# Autodesk Inventor assembly: Wheel Assembly
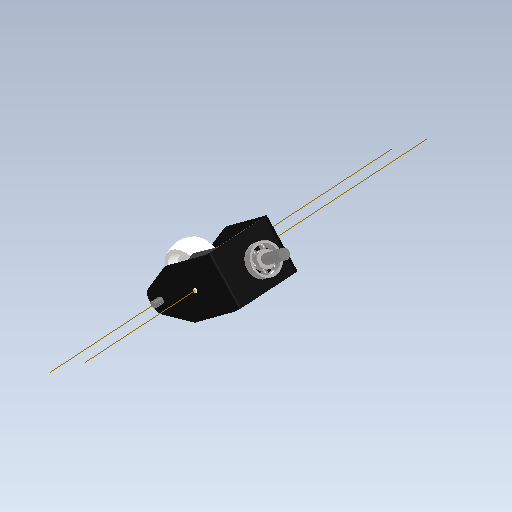
[picture p0: Inventor's stored thumbnail of the model, 512x512]
Saved by Autodesk Inventor 2020 (Build 240168000, 168)
## iProperties
Created: 2022-07-01
Part Number: Wheel Assembly
Document SubType Name: Assembly
Designer: karimi2
Author: karimi2
## Documents named in this file (14)
- C:\Users\karimi2\Documents\PROJECT\src\Wheel Assembly.iam
- C:\Users\karimi2\Documents\PROJECT\src\New frame.ipt
- C:\Users\karimi2\Documents\PROJECT\src\wheelshaftGenerated.ipt
- C:\Users\karimi2\Documents\PROJECT\src\casterwheel.ipt
- C:\Users\karimi2\Documents\PROJECT\src\Bearing M8.iam
- C:\Users\karimi2\Documents\PROJECT\src\Shaft 8mm.ipt
- C:\Users\karimi2\Documents\PROJECT\src\motorAssembly.iam
- C:\Users\karimi2\Documents\PROJECT\src\Wheel Assembly\Design Accelerator\Synchronous Belts Transmission2.iam
- C:\Users\karimi2\Documents\PROJECT\src\Wheel Assembly\AIP\FEA\e1f7mqq1s.fins
- C:\Users\karimi2\Documents\PROJECT\src\Wheel Assembly\AIP\FEA\e1f7mqq1s.fsat
- C:\Users\karimi2\Documents\PROJECT\src\Wheel Assembly\AIP\FEA\e1f7mqq1s.ftes
- C:\Users\karimi2\Documents\PROJECT\src\Wheel Assembly\AIP\FEA\e1f7mqq1s.fwiz
- C:\Users\karimi2\Documents\PROJECT\src\Wheel Assembly\AIP\FEA\e1f7mqq4g.fmsh
- C:\Users\karimi2\Documents\PROJECT\src\Wheel Assembly\AIP\FEA\e1f7mqq4h.fres
## Components (7 placed, 7 different names)
1. New frame:1 — Mate:3, Mate:4, Mate:6, Rigid:3, Flush:1, Mate:14
2. Shaft:1 — Mate:3, Mate:4, Mate:5, Mate:17
3. casterwheel:1 — Mate:5, Mate:6
4. Shaft 8mm:1 — Rigid:3, Rotational:1, Mate:18
5. Bearing M8:1 [sub-assembly] — Rotational:1, Mate:18
6. motorAssembly:1 [sub-assembly] — Flush:1, Mate:14, Mate:15, Mate:16
7. Synchronous Belts Transmission:1 [sub-assembly] — Mate:15, Mate:16, Mate:17
## Relationships (12: Mate 9, WeldJoint 1, RevoluteJoint 1, Flush 1)
- Mate:3: New frame:1 ↔ Shaft:1
- Mate:4 (-9 mm): New frame:1 ↔ Shaft:1
- Mate:5: Shaft:1 ↔ casterwheel:1
- Mate:6 (10 mm): New frame:1 ↔ casterwheel:1
- Rigid:3 [WeldJoint]: New frame:1 ↔ Shaft 8mm:1
- Rotational:1 [RevoluteJoint] (-23 mm): Shaft 8mm:1 ↔ Bearing M8:1
- Flush:1 (-8.25 mm): New frame:1 ↔ motorAssembly:1
- Mate:14: New frame:1 ↔ motorAssembly:1
- Mate:15: motorAssembly:1 ↔ Synchronous Belts Transmission:1
- Mate:16 (2.5 mm): motorAssembly:1 ↔ Synchronous Belts Transmission:1
- Mate:17: Shaft:1 ↔ Synchronous Belts Transmission:1
- Mate:18: Shaft 8mm:1 ↔ Bearing M8:1
## Named parameters: sa_0 = 10000
note: some values were not read from the file. Shown as the stored number, unit unknown: "sa_0".
